# Autodesk Inventor assembly: Assembly1
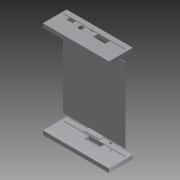
[picture p0: Inventor's stored thumbnail of the model, 180x180]
Saved by Autodesk Inventor 2012 (Build 160160000, 160)
## iProperties
Created: 2017-04-26
Part Number: Assembly1
Document SubType Name: Assembly
Designer: Brandon
Author: Brandon
## Documents named in this file (10)
- C:\Users\Brandon\Dropbox\Admiral Instruments Dropbox\Squidstat Plus 2.0 (single channel, with EIS)\Enclosure\Assembly1.iam
- C:\Users\Brandon\Dropbox\Admiral Instruments Dropbox\Squidstat Plus 2.0 (single channel, with EIS)\Enclosure\PCB.ipt
- C:\Users\Brandon\Dropbox\Admiral Instruments Dropbox\Squidstat Plus 2.0 (single channel, with EIS)\Enclosure\LED on indicator.ipt
- C:\Users\Brandon\Dropbox\Admiral Instruments Dropbox\Squidstat Plus 2.0 (single channel, with EIS)\Enclosure\DB15 connector.ipt
- C:\Users\Brandon\Dropbox\Admiral Instruments Dropbox\Squidstat Plus 2.0 (single channel, with EIS)\Enclosure\USB A block.ipt
- C:\Users\Brandon\Dropbox\Admiral Instruments Dropbox\Squidstat Plus 2.0 (single channel, with EIS)\Enclosure\Grounded banana jack.ipt
- C:\Users\Brandon\Dropbox\Admiral Instruments Dropbox\Squidstat Plus 2.0 (single channel, with EIS)\Enclosure\Slide switch.ipt
- C:\Users\Brandon\Dropbox\Admiral Instruments Dropbox\Squidstat Plus 2.0 (single channel, with EIS)\Enclosure\DB9 connector.ipt
- C:\Users\Brandon\Dropbox\Admiral Instruments Dropbox\Squidstat Plus 2.0 (single channel, with EIS)\Enclosure\back cover.ipt
- C:\Users\Brandon\Dropbox\Admiral Instruments Dropbox\Squidstat Plus 2.0 (single channel, with EIS)\Enclosure\front cover.ipt
## Components (9 placed, 9 different names)
1. PCB:1 — Flush:1, Insert:1, Flush:1, Insert:2, Insert:4, Angle:4, Mate:1, Insert:5, Angle:5, Insert:6, Angle:6, Flush:5, Insert:7
2. LED on indicator:1 — Flush:1, Insert:1, Angle:3
3. DB15 connector:1 — Flush:1, Insert:2, Angle:2
4. Grounded banana jack:1 — Insert:4, Angle:4
5. Slide switch:1 — Mate:1, Insert:5, Angle:5
6. DB9 connector:1 — Insert:6, Angle:6
7. back cover:1 — Mate:3, Mate:4, Flush:4, Flush:5
8. front cover:1 — Flush:3, Mate:2, Flush:4
9. USB A block:1 — Insert:7, Angle:7
## Relationships (21: Insert 6, Angle 6, Flush 5, Mate 4)
- Flush:1: PCB:1 ↔ LED on indicator:1
- Insert:1: PCB:1 ↔ LED on indicator:1
- Flush:1: PCB:1 ↔ DB15 connector:1
- Insert:2: PCB:1 ↔ DB15 connector:1
- Angle:2 (180 deg): DB15 connector:1
- Angle:3 (180 deg): LED on indicator:1
- Insert:4: PCB:1 ↔ Grounded banana jack:1
- Angle:4 (0 deg): PCB:1 ↔ Grounded banana jack:1
- Mate:1: PCB:1 ↔ Slide switch:1
- Insert:5: PCB:1 ↔ Slide switch:1
- Angle:5 (0 deg): PCB:1 ↔ Slide switch:1
- Insert:6: PCB:1 ↔ DB9 connector:1
- Angle:6 (0 deg): PCB:1 ↔ DB9 connector:1
- Flush:3 (114.3 mm): front cover:1
- Mate:2: front cover:1
- Mate:3 (114.3 mm): back cover:1
- Mate:4: back cover:1
- Flush:4: back cover:1 ↔ front cover:1
- Flush:5 (12.7 mm): PCB:1 ↔ back cover:1
- Insert:7: PCB:1 ↔ USB A block:1
- Angle:7 (180 deg): USB A block:1
